# Autodesk Inventor assembly: Assembly
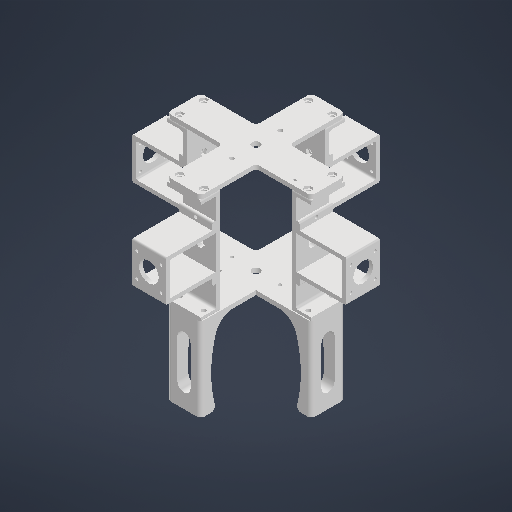
[picture p0: Inventor's stored thumbnail of the model, 512x512]
Saved by Autodesk Inventor 2026 (Build 300175050, 175E)
## iProperties
Created: 2025-10-07
Part Number: Assembly
Document SubType Name: Assembly
Designer: aduwa
Author: aduwa
## Documents named in this file (5)
- C:\Users\aduwa\OneDrive\Documents\PROJECTS\data\2025\CAPSTONE\V4.1\STL\Assembly.iam
- C:\Users\aduwa\OneDrive\Documents\PROJECTS\data\2025\CAPSTONE\V4.1\baseMount.ipt
- C:\Users\aduwa\OneDrive\Documents\PROJECTS\data\2025\CAPSTONE\V4.1\sideMount.ipt
- C:\Users\aduwa\OneDrive\Documents\PROJECTS\data\2025\CAPSTONE\V4.1\topMount.ipt
- C:\Users\aduwa\OneDrive\Documents\PROJECTS\data\2025\CAPSTONE\V4.1\motorMount.ipt
## Components (10 placed, 4 different names)
1. baseMount:1 — Mate:1, Mate:2, Mate:3, Mate:4, Mate:5, Mate:6, Mate:7, Mate:8, Mate:9, Mate:10, Mate:11, Mate:12, Mate:13
2. sideMount:1 — Mate:1, Mate:2, Mate:3, Mate:19, Mate:20
3. sideMount:2 — Mate:7, Mate:8, Mate:9, Mate:15, Mate:17, Mate:18
4. sideMount:3 — Mate:10, Mate:11, Mate:12, Mate:23, Mate:24
5. sideMount:4 — Mate:4, Mate:5, Mate:6, Mate:14, Mate:16, Mate:21, Mate:22
6. topMount:1 — Mate:13, Mate:14, Mate:15, Mate:16
7. motorMount:1 — Mate:17, Mate:18
8. motorMount:2 — Mate:19, Mate:20
9. motorMount:3 — Mate:21, Mate:22
10. motorMount:4 — Mate:23, Mate:24
## Relationships (24: Mate 24)
- Mate:1: baseMount:1 ↔ sideMount:1
- Mate:2: baseMount:1 ↔ sideMount:1
- Mate:3: baseMount:1 ↔ sideMount:1
- Mate:4: baseMount:1 ↔ sideMount:4
- Mate:5: baseMount:1 ↔ sideMount:4
- Mate:6: baseMount:1 ↔ sideMount:4
- Mate:7: baseMount:1 ↔ sideMount:2
- Mate:8: baseMount:1 ↔ sideMount:2
- Mate:9: baseMount:1 ↔ sideMount:2
- Mate:10: baseMount:1 ↔ sideMount:3
- Mate:11: baseMount:1 ↔ sideMount:3
- Mate:12: baseMount:1 ↔ sideMount:3
- Mate:13: baseMount:1 ↔ topMount:1
- Mate:14: sideMount:4 ↔ topMount:1
- Mate:15: sideMount:2 ↔ topMount:1
- Mate:16: sideMount:4 ↔ topMount:1
- Mate:17: sideMount:2 ↔ motorMount:1
- Mate:18: sideMount:2 ↔ motorMount:1
- Mate:19: sideMount:1 ↔ motorMount:2
- Mate:20: sideMount:1 ↔ motorMount:2
- Mate:21: sideMount:4 ↔ motorMount:3
- Mate:22: sideMount:4 ↔ motorMount:3
- Mate:23: sideMount:3 ↔ motorMount:4
- Mate:24: sideMount:3 ↔ motorMount:4
